# Autodesk Inventor assembly: 20-J2
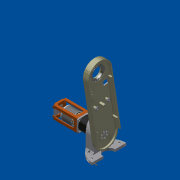
[picture p0: Inventor's stored thumbnail of the model, 180x180]
Saved by Autodesk Inventor 2018 (Build 220112000, 112)
## iProperties
Created: 2020-01-14
Part Number: 20-J2
Document SubType Name: Assembly
Designer: Bunny320
Author: Bunny320
## Documents named in this file (10)
- D:\Seerosenstr\sechs\4-CAD\20-J2.iam
- D:\Seerosenstr\sechs\4-CAD\201-flange-with motor.ipt
- D:\Seerosenstr\sechs\4-CAD\standardParts\61807-2RS1\61807-2RS1.iam
- D:\Seerosenstr\sechs\4-CAD\motor unit.iam
- D:\Seerosenstr\sechs\4-CAD\203-link left.ipt
- C:\Users\mo\Documents\Inventor\Content Center Files\R2018\en-US\ISO 4762(1)\DIN EN ISO 4762 - M3 x 12.ipt
- C:\Users\mo\Documents\Inventor\Content Center Files\R2018\en-US\ISO 4762(1)\DIN EN ISO 4762 - M3 x 20.ipt
- C:\Users\Bunny320\Documents\Inventor\Content Center Files\R2018\en-US\DIN EN ISO 4032\DIN EN ISO 4032 - M3.ipt
- D:\Seerosenstr\sechs\4-CAD\standardParts\Pololu mounting hub\pololu-universal-aluminum-mounting-hub-for-8mm-shaft-m3-holes.ipt
- D:\Seerosenstr\sechs\4-CAD\standardParts\W 619_4-2Z\W 619_4-2Z.iam
## Components (14 placed, 9 different names)
1. 201-flange-with motor:1 — Flush:1, Flush:2, Flush:3, Mate:3, Mate:7, Mate:8, Mate:9, Mate:31, Mate:32, Mate:33, Mate:34, Mate:35, Mate:36, Mate:37, Mate:38, Mate:39, Mate:40, Mate:48
2. 61807-2RS1:1 [sub-assembly] — Mate:3, Mate:48, Mate:49, Mate:53
3. motor unit:1 [sub-assembly] — Mate:7, Mate:8, Mate:9
4. 61807-2RS1:3 [sub-assembly] — Mate:54, Mate:55
5. DIN EN ISO 4762 M3 x 12:4 — Mate:31, Mate:32
6. DIN EN ISO 4762 M3 x 12:5 — Mate:33, Mate:34
7. DIN EN ISO 4762 M3 x 12:6 — Mate:35, Mate:36
8. DIN EN ISO 4762 M3 x 12:7 — Mate:37, Mate:38
9. DIN EN ISO 4762 M3 x 20:1 — Mate:39, Mate:40
10. DIN EN ISO 4032 M3:1
11. pololu-universal-aluminum-mounting-hub-for-8mm-shaft-m3-holes:1 — Mate:50, Mate:51, Mate:52
12. 203-link left:1 — Mate:49, Mate:50, Mate:51, Mate:52, Mate:53, Mate:54, Mate:55, Mate:56, Mate:57, Mate:58, Mate:59
13. W 619_4-2Z:1 [sub-assembly] — Mate:56, Mate:59
14. W 619_4-2Z:2 [sub-assembly] — Mate:57, Mate:58
## Relationships (29: Mate 26, Flush 3)
- Flush:1: 201-flange-with motor:1
- Flush:2: 201-flange-with motor:1
- Flush:3: 201-flange-with motor:1
- Mate:3: 201-flange-with motor:1 ↔ 61807-2RS1:1
- Mate:7: 201-flange-with motor:1 ↔ motor unit:1
- Mate:8: 201-flange-with motor:1 ↔ motor unit:1
- Mate:9: 201-flange-with motor:1 ↔ motor unit:1
- Mate:31: 201-flange-with motor:1 ↔ DIN EN ISO 4762 M3 x 12:4
- Mate:32: 201-flange-with motor:1 ↔ DIN EN ISO 4762 M3 x 12:4
- Mate:33: 201-flange-with motor:1 ↔ DIN EN ISO 4762 M3 x 12:5
- Mate:34: 201-flange-with motor:1 ↔ DIN EN ISO 4762 M3 x 12:5
- Mate:35: 201-flange-with motor:1 ↔ DIN EN ISO 4762 M3 x 12:6
- Mate:36: 201-flange-with motor:1 ↔ DIN EN ISO 4762 M3 x 12:6
- Mate:37: 201-flange-with motor:1 ↔ DIN EN ISO 4762 M3 x 12:7
- Mate:38: 201-flange-with motor:1 ↔ DIN EN ISO 4762 M3 x 12:7
- Mate:39: 201-flange-with motor:1 ↔ DIN EN ISO 4762 M3 x 20:1
- Mate:40: 201-flange-with motor:1 ↔ DIN EN ISO 4762 M3 x 20:1
- Mate:48: 201-flange-with motor:1 ↔ 61807-2RS1:1
- Mate:49: 61807-2RS1:1 ↔ 203-link left:1
- Mate:50: pololu-universal-aluminum-mounting-hub-for-8mm-shaft-m3-holes:1 ↔ 203-link left:1
- Mate:51: pololu-universal-aluminum-mounting-hub-for-8mm-shaft-m3-holes:1 ↔ 203-link left:1
- Mate:52: pololu-universal-aluminum-mounting-hub-for-8mm-shaft-m3-holes:1 ↔ 203-link left:1
- Mate:53: 61807-2RS1:1 ↔ 203-link left:1
- Mate:54: 61807-2RS1:3 ↔ 203-link left:1
- Mate:55: 61807-2RS1:3 ↔ 203-link left:1
- Mate:56: 203-link left:1 ↔ W 619_4-2Z:1
- Mate:57: 203-link left:1 ↔ W 619_4-2Z:2
- Mate:58: 203-link left:1 ↔ W 619_4-2Z:2
- Mate:59: 203-link left:1 ↔ W 619_4-2Z:1
